# Autodesk Inventor assembly: BatteryPack
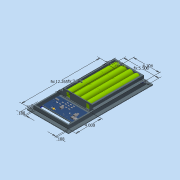
[picture p0: Inventor's stored thumbnail of the model, 180x180]
Saved by Autodesk Inventor 2015 (Build 190159000, 159)
## iProperties
Created: 2015-10-11
Part Number: BatteryPack
Document SubType Name: Assembly
Designer: Raphael
Author: Raphael
## Documents named in this file (4)
- \\psf\Home\Documents\electric-skateboard\CAD\BatteryPack.iam
- \\psf\Home\Documents\electric-skateboard\CAD\BatteryBox.ipt
- \\psf\Home\Documents\electric-skateboard\CAD\BMS.ipt
- \\psf\Home\Documents\electric-skateboard\CAD\26650.ipt
## Components (14 placed, 3 different names)
1. BatteryBox:1 — Mate:1, Flush:1, Mate:2, Mate:3, Mate:4, Mate:9, Mate:10, Mate:15, Mate:16, Mate:21, Mate:22, Mate:24
2. BMS:1 — Mate:1, Flush:1, Mate:2
3. 26650:1 — Mate:3, Mate:4, Mate:5, Mate:6
4. 26650:2 — Mate:5, Mate:6, Mate:7, Mate:8
5. 26650:3 — Mate:7, Mate:8
6. 26650:4 — Mate:9, Mate:10, Mate:11, Mate:12
7. 26650:5 — Mate:11, Mate:12, Mate:13, Mate:14
8. 26650:6 — Mate:13, Mate:14
9. 26650:7 — Mate:15, Mate:16, Mate:17, Mate:18
10. 26650:8 — Mate:17, Mate:18, Mate:19, Mate:20
11. 26650:9 — Mate:19, Mate:20
12. 26650:10 — Mate:21, Mate:22, Mate:23
13. 26650:11 — Mate:23, Mate:24, Mate:25, Mate:26
14. 26650:12 — Mate:25, Mate:26
## Relationships (27: Mate 26, Flush 1)
- Mate:1: BatteryBox:1 ↔ BMS:1
- Flush:1: BatteryBox:1 ↔ BMS:1
- Mate:2 (1.5875 mm): BatteryBox:1 ↔ BMS:1
- Mate:3 (0.127 mm): BatteryBox:1 ↔ 26650:1
- Mate:4: BatteryBox:1 ↔ 26650:1
- Mate:5 (0.254 mm): 26650:1 ↔ 26650:2
- Mate:6: 26650:1 ↔ 26650:2
- Mate:7 (0.254 mm): 26650:2 ↔ 26650:3
- Mate:8: 26650:2 ↔ 26650:3
- Mate:9 (0.127 mm): BatteryBox:1 ↔ 26650:4
- Mate:10: BatteryBox:1 ↔ 26650:4
- Mate:11 (0.254 mm): 26650:4 ↔ 26650:5
- Mate:12: 26650:4 ↔ 26650:5
- Mate:13 (0.254 mm): 26650:5 ↔ 26650:6
- Mate:14: 26650:5 ↔ 26650:6
- Mate:15 (0.127 mm): BatteryBox:1 ↔ 26650:7
- Mate:16: BatteryBox:1 ↔ 26650:7
- Mate:17 (0.254 mm): 26650:7 ↔ 26650:8
- Mate:18: 26650:7 ↔ 26650:8
- Mate:19 (0.254 mm): 26650:8 ↔ 26650:9
- Mate:20: 26650:8 ↔ 26650:9
- Mate:21 (0.127 mm): BatteryBox:1 ↔ 26650:10
- Mate:22: BatteryBox:1 ↔ 26650:10
- Mate:23 (0.254 mm): 26650:10 ↔ 26650:11
- Mate:24: BatteryBox:1 ↔ 26650:11
- Mate:25 (0.254 mm): 26650:11 ↔ 26650:12
- Mate:26: 26650:11 ↔ 26650:12
